# Autodesk Inventor assembly: ToASI-2
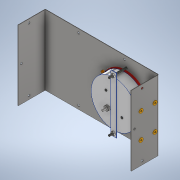
[picture p0: Inventor's stored thumbnail of the model, 180x180]
Saved by Autodesk Inventor 2020.3 (Build 243373000, 373)
## iProperties
Created: 2020-07-31
Part Number: ToASI-2
Document SubType Name: Assembly
Designer: Bruno
Author: Bruno
## Documents named in this file (6)
- C:\Users\Bruno\Desktop\Github\CAD\Inventor\For ASI\ToASI-2.iam
- C:\Users\Bruno\Desktop\Github\CAD\Inventor\For ASI\ToASI-0B.iam
- C:\Users\Bruno\Desktop\Github\CAD\Inventor\For ASI\ToASI-1.iam
- C:\Users\Bruno\Desktop\Github\CAD\Inventor\Heater-Box\Box-Disk\DIN912 M4x0.7x40-8.8 socket head screw.ipt
- C:\Users\Bruno\Desktop\Github\CAD\Inventor\Heater-Box\Box-Disk\Heater Fixing Bar.ipt
- C:\Users\Bruno\Desktop\Github\CAD\Inventor\Heater-Box\Box-Disk\DIN934-M4 nut.ipt
## Components (7 placed, 5 different names)
1. ToASI-0B:1 [sub-assembly] — Cylindrical:1, Cylindrical:2, Cylindrical:3, Angle:1
2. ToASI-1:1 [sub-assembly] — Cylindrical:1, Mate:1
3. DIN912 M4x0.7x40-8.8 socket head screw:1 — Cylindrical:2
4. DIN912 M4x0.7x40-8.8 socket head screw:2 — Cylindrical:3, Cylindrical:4
5. Heater Fixing Bar:1 — Mate:1, Cylindrical:4, Angle:1, Cylindrical:5, Cylindrical:6
6. DIN934-M4 nut:1 — Cylindrical:5
7. DIN934-M4 nut:2 — Cylindrical:6
## Relationships (8: CylindricalJoint 6, Mate 1, Angle 1)
- Cylindrical:1: ToASI-0B:1 ↔ ToASI-1:1
- Cylindrical:2: ToASI-0B:1 ↔ DIN912 M4x0.7x40-8.8 socket head screw:1
- Cylindrical:3: ToASI-0B:1 ↔ DIN912 M4x0.7x40-8.8 socket head screw:2
- Mate:1: ToASI-1:1 ↔ Heater Fixing Bar:1
- Cylindrical:4: DIN912 M4x0.7x40-8.8 socket head screw:2 ↔ Heater Fixing Bar:1
- Angle:1 (0 deg): ToASI-0B:1 ↔ Heater Fixing Bar:1
- Cylindrical:5: Heater Fixing Bar:1 ↔ DIN934-M4 nut:1
- Cylindrical:6: Heater Fixing Bar:1 ↔ DIN934-M4 nut:2
